# Autodesk Inventor assembly: Assembly2
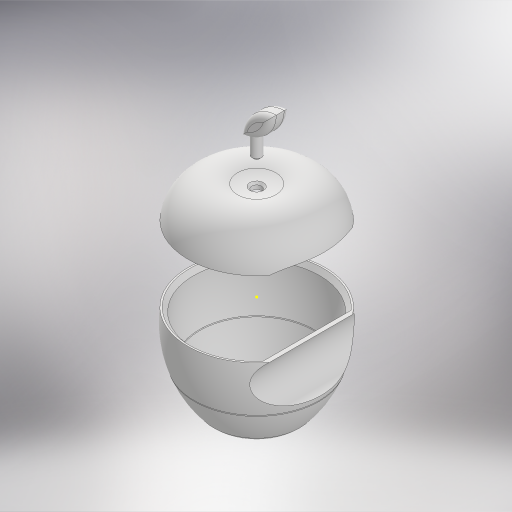
[picture p0: Inventor's stored thumbnail of the model, 512x512]
Saved by Autodesk Inventor 2024 (Build 280153000, 153)
## iProperties
Created: 2023-11-01
Part Number: Assembly2
Document SubType Name: Assembly
Designer: SSAFY
Author: SSAFY
## Documents named in this file (4)
- C:\Users\SSAFY\Desktop\TIL\3D\20231101\Assembly2.iam
- C:\Users\SSAFY\Desktop\TIL\3D\20231101\Apple_logo_red.ipt
- C:\Users\SSAFY\Desktop\TIL\3D\20231101\Apple_logo_red2.ipt
- C:\Users\SSAFY\Desktop\TIL\3D\20231101\Apple_logo_black.ipt
## Components (3 placed, 3 different names)
1. Apple_logo_red:2 — Mate:1, Flush:1, Flush:2
2. Apple_logo_red2:1 — Flush:3, Flush:4, Mate:2
3. Apple_logo_black:1 — Mate:2, Flush:5, Flush:6
## Relationships (8: Flush 6, Mate 2)
- Mate:1: Apple_logo_red:2
- Flush:1: Apple_logo_red:2
- Flush:2: Apple_logo_red:2
- Flush:3: Apple_logo_red2:1
- Flush:4: Apple_logo_red2:1
- Mate:2: Apple_logo_red2:1 ↔ Apple_logo_black:1
- Flush:5: Apple_logo_black:1
- Flush:6: Apple_logo_black:1
